# Autodesk Inventor assembly: daVinci_head_motorizedSled_ToolFixation
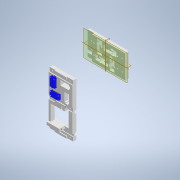
[picture p0: Inventor's stored thumbnail of the model, 180x180]
Saved by Autodesk Inventor 2022 (Build 260153000, 153)
## iProperties
Created: 2022-08-16
Part Number: daVinci_head_motorizedSled_ToolFixation
Document SubType Name: Assembly
Designer: alexw
Author: alexw
## Documents named in this file (4)
- C:\Users\alexw\Documents\Inventor\Projects\03_CurrentProjects\MasterThesis\PSM_V1_Rillenkugellager\Ueberarbeiteter DaVincikopf\daVinci_head_motorizedSled_ToolFixation.iam
- C:\Users\alexw\Documents\Inventor\Projects\03_CurrentProjects\MasterThesis\PSM_V1_Rillenkugellager\Ueberarbeiteter DaVincikopf\Fuehrungsgrundplatte_V3.ipt
- C:\Users\alexw\Documents\Inventor\Projects\03_CurrentProjects\MasterThesis\PSM_V1_Rillenkugellager\Ueberarbeiteter DaVincikopf\Oberteil_servoplatte.ipt
- C:\Users\alexw\Documents\Inventor\Projects\03_CurrentProjects\MasterThesis\PSM_V1_Rillenkugellager\Ueberarbeiteter DaVincikopf\sg90-micro-servo-9g-tower-pro-1.snapshot.3\SG90 - Micro Servo 9g - Tower Pro.iam
## Components (4 placed, 3 different names)
1. Fuehrungsgrundplatte_V3:1 — Fluchtend:1, Fluchtend:2, Fluchtend:3, Fluchtend:4, Passend:1, Passend:2, Passend:3, Passend:4, Passend:5, Passend:6
2. Oberteil_servoplatte:1
3. SG90 - Micro Servo 9g - Tower Pro:1 [sub-assembly] — Passend:1, Passend:2, Passend:3
4. SG90 - Micro Servo 9g - Tower Pro:2 [sub-assembly] — Passend:4, Passend:5, Passend:6
## Relationships (10: Mate 6, Flush 4)
- Fluchtend:1 [Flush]: Fuehrungsgrundplatte_V3:1
- Fluchtend:2 [Flush]: Fuehrungsgrundplatte_V3:1
- Fluchtend:3 [Flush]: Fuehrungsgrundplatte_V3:1
- Fluchtend:4 [Flush]: Fuehrungsgrundplatte_V3:1
- Passend:1 [Mate]: Fuehrungsgrundplatte_V3:1 ↔ SG90 - Micro Servo 9g - Tower Pro:1
- Passend:2 [Mate]: Fuehrungsgrundplatte_V3:1 ↔ SG90 - Micro Servo 9g - Tower Pro:1
- Passend:3 [Mate]: Fuehrungsgrundplatte_V3:1 ↔ SG90 - Micro Servo 9g - Tower Pro:1
- Passend:4 [Mate]: Fuehrungsgrundplatte_V3:1 ↔ SG90 - Micro Servo 9g - Tower Pro:2
- Passend:5 [Mate]: Fuehrungsgrundplatte_V3:1 ↔ SG90 - Micro Servo 9g - Tower Pro:2
- Passend:6 [Mate]: Fuehrungsgrundplatte_V3:1 ↔ SG90 - Micro Servo 9g - Tower Pro:2
